# Autodesk Inventor assembly: metabotV2
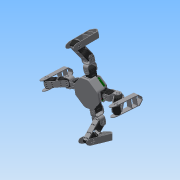
[picture p0: Inventor's stored thumbnail of the model, 180x180]
Saved by Autodesk Inventor 2015 (Build 190159000, 159)
## iProperties
Created: 2014-03-07
Part Number: metabotV2
Document SubType Name: Assembly
Designer: Grégoire
Author: Grégoire
## Documents named in this file (14)
- C:\Users\Gregwar\Desktop\Metabot\3d\autodesk\metabotV2.iam
- C:\Users\Gregwar\Desktop\Metabot\3d\autodesk\models\motor.ipt
- C:\Users\Gregwar\Desktop\Metabot\3d\autodesk\models\arm.ipt
- C:\Users\Gregwar\Desktop\Metabot\3d\autodesk\models\counter_arm.ipt
- C:\Users\Gregwar\Desktop\Metabot\3d\autodesk\parts\u.ipt
- C:\Users\Gregwar\Desktop\Metabot\3d\autodesk\parts\side.ipt
- C:\Users\Gregwar\Desktop\Metabot\3d\autodesk\parts\leg.ipt
- C:\Users\Gregwar\Desktop\Metabot\3d\autodesk\parts\bottom.ipt
- C:\Users\Gregwar\Desktop\Metabot\3d\autodesk\renfort.ipt
- C:\Users\Gregwar\Desktop\Metabot\3d\autodesk\models\x_board.ipt
- C:\Users\Gregwar\Desktop\Metabot\3d\autodesk\fix_top.ipt
- C:\Users\Gregwar\Desktop\Metabot\3d\autodesk\parts\magnet.ipt
- C:\Users\Gregwar\Desktop\Metabot\3d\autodesk\parts\head.ipt
- C:\Users\Gregwar\Desktop\Metabot\3d\autodesk\parts\top.ipt
## Components (66 placed, 13 different names)
1. motor:4 — Affleurement:2, Affleurement:4, Affleurement:5, Placage:211, Placage:217, Placage:218
2. arm:4 — Placage:167
3. counter_arm:4
4. u:3
5. u:4 — Placage:167
6. motor:5
7. arm:5
8. counter_arm:5
9. side:3
10. side:4
11. motor:6
12. arm:6
13. counter_arm:6
14. leg:2
15. motor:7 — Affleurement:3, Affleurement:4, Placage:215, Placage:216, Placage:223, Placage:224, Placage:225, Placage:241, Placage:242, Placage:243
16. arm:7
17. counter_arm:7 — Placage:168
18. u:5
19. u:6 — Placage:168
20. motor:8
21. arm:8
22. counter_arm:8
23. side:5
24. side:6
25. motor:9
26. arm:9
27. counter_arm:9
28. leg:3
29. motor:10 — Affleurement:1, Affleurement:2, Affleurement:5, Placage:197, Placage:212, Placage:219
30. arm:10
31. counter_arm:10 — Placage:169
32. u:7
33. u:8 — Placage:169
34. motor:11
35. arm:11
36. counter_arm:11
37. side:7
38. side:8
39. motor:12
40. arm:12
41. counter_arm:12
42. leg:4
43. renfort:1 — Placage:197
44. x_board:1 — Placage:221, Placage:222, Placage:226
45. bottom:1 — Placage:211, Placage:212, Placage:213, Placage:214, Placage:215, Placage:216, Placage:217, Placage:218, Placage:219, Placage:221, Placage:222, Placage:226
46. fix_top:1 — Placage:223, Placage:224, Placage:225, Placage:227, Placage:228, Placage:229, Placage:230, Placage:231, Placage:232, Placage:233, Placage:234, Placage:235, Placage:236, Placage:237, Placage:238, Placage:240
47. magnet:1 — Placage:227, Placage:228, Placage:229, Affleurement:6, Placage:244, Placage:245
48. magnet:2 — Placage:230, Placage:231, Placage:232, Affleurement:8, Placage:248, Placage:249, Placage:253
49. magnet:3 — Placage:233, Placage:234, Placage:235, Affleurement:7, Placage:246, Placage:247
50. magnet:4 — Placage:236, Placage:237, Placage:238, Placage:239, Affleurement:6, Affleurement:7, Affleurement:8, Placage:250, Placage:251
51. head:2 — Placage:239, Placage:240, Placage:252, Placage:254
52. top:1 — Placage:241, Placage:242, Placage:243, Placage:244, Placage:245, Placage:246, Placage:247, Placage:248, Placage:249, Placage:250, Placage:251, Placage:252, Placage:253, Placage:254
53. u:1 — Placage:7, Placage:8, Placage:9, Placage:14, Placage:15
54. u:2 — Placage:6, Placage:7, Placage:8, Placage:9, Placage:164, Placage:166
55. side:1 — Placage:19, Placage:20, Placage:21, Placage:26, Placage:27, Placage:28
56. side:2 — Placage:16, Placage:17, Placage:18
57. leg:1 — Placage:29, Placage:30
58. motor:1 — Placage:1, Placage:2, Placage:3, Placage:4, Affleurement:1, Affleurement:3, Placage:213, Placage:214
59. arm:1 — Placage:3, Placage:4, Placage:6, Placage:166
60. counter_arm:1 — Placage:1, Placage:2, Placage:164
61. motor:2 — Placage:16, Placage:17, Placage:18, Placage:19, Placage:20, Placage:21
62. arm:2 — Placage:15
63. counter_arm:2 — Placage:14
64. motor:3 — Placage:26, Placage:27, Placage:28
65. arm:3 — Placage:29, Placage:30
66. counter_arm:3
## Relationships (173: Mate 165, Flush 8)
- Placage:1 [Mate]: motor:1 ↔ counter_arm:1
- Placage:2 [Mate]: motor:1 ↔ counter_arm:1
- Placage:3 [Mate]: motor:1 ↔ arm:1
- Placage:4 [Mate]: motor:1 ↔ arm:1
- Placage:6 [Mate]: u:2 ↔ arm:1
- Placage:7 [Mate]: u:1 ↔ u:2
- Placage:8 [Mate]: u:1 ↔ u:2
- Placage:9 [Mate]: u:1 ↔ u:2
- [Mate]: motor:2 ↔ counter_arm:2
- [Mate]: motor:2 ↔ counter_arm:2
- [Mate]: motor:2 ↔ arm:2
- [Mate]: motor:2 ↔ arm:2
- Placage:14 [Mate]: u:1 ↔ counter_arm:2
- Placage:15 [Mate]: u:1 ↔ arm:2
- Placage:16 [Mate]: side:2 ↔ motor:2
- Placage:17 [Mate]: side:2 ↔ motor:2
- Placage:18 [Mate]: side:2 ↔ motor:2
- Placage:19 [Mate]: side:1 ↔ motor:2
- Placage:20 [Mate]: side:1 ↔ motor:2
- Placage:21 [Mate]: side:1 ↔ motor:2
- [Mate]: motor:3 ↔ counter_arm:3
- [Mate]: motor:3 ↔ counter_arm:3
- [Mate]: motor:3 ↔ arm:3
- [Mate]: motor:3 ↔ arm:3
- Placage:26 [Mate]: side:1 ↔ motor:3
- Placage:27 [Mate]: side:1 ↔ motor:3
- Placage:28 [Mate]: side:1 ↔ motor:3
- Placage:29 [Mate]: leg:1 ↔ arm:3
- Placage:30 [Mate]: leg:1 ↔ arm:3
- [Mate]: motor:4 ↔ counter_arm:4
- [Mate]: motor:4 ↔ counter_arm:4
- [Mate]: motor:4 ↔ arm:4
- [Mate]: motor:4 ↔ arm:4
- [Mate]: arm:4 ↔ u:4
- [Mate]: u:3 ↔ u:4
- [Mate]: u:3 ↔ u:4
- [Mate]: u:3 ↔ u:4
- [Mate]: motor:5 ↔ counter_arm:5
- [Mate]: motor:5 ↔ counter_arm:5
- [Mate]: motor:5 ↔ arm:5
- [Mate]: motor:5 ↔ arm:5
- [Mate]: u:3 ↔ counter_arm:5
- [Mate]: u:3 ↔ arm:5
- [Mate]: motor:5 ↔ side:4
- [Mate]: motor:5 ↔ side:4
- [Mate]: motor:5 ↔ side:4
- [Mate]: motor:5 ↔ side:3
- [Mate]: motor:5 ↔ side:3
- [Mate]: motor:5 ↔ side:3
- [Mate]: motor:6 ↔ counter_arm:6
- [Mate]: motor:6 ↔ counter_arm:6
- [Mate]: motor:6 ↔ arm:6
- [Mate]: motor:6 ↔ arm:6
- [Mate]: side:3 ↔ motor:6
- [Mate]: side:3 ↔ motor:6
- [Mate]: side:3 ↔ motor:6
- [Mate]: arm:6 ↔ leg:2
- [Mate]: arm:6 ↔ leg:2
- [Mate]: motor:7 ↔ counter_arm:7
- [Mate]: motor:7 ↔ counter_arm:7
- [Mate]: motor:7 ↔ arm:7
- [Mate]: motor:7 ↔ arm:7
- [Mate]: arm:7 ↔ u:6
- [Mate]: u:5 ↔ u:6
- [Mate]: u:5 ↔ u:6
- [Mate]: u:5 ↔ u:6
- [Mate]: motor:8 ↔ counter_arm:8
- [Mate]: motor:8 ↔ counter_arm:8
- [Mate]: motor:8 ↔ arm:8
- [Mate]: motor:8 ↔ arm:8
- [Mate]: u:5 ↔ counter_arm:8
- [Mate]: u:5 ↔ arm:8
- [Mate]: motor:8 ↔ side:6
- [Mate]: motor:8 ↔ side:6
- [Mate]: motor:8 ↔ side:6
- [Mate]: motor:8 ↔ side:5
- [Mate]: motor:8 ↔ side:5
- [Mate]: motor:8 ↔ side:5
- [Mate]: motor:9 ↔ counter_arm:9
- [Mate]: motor:9 ↔ counter_arm:9
- [Mate]: motor:9 ↔ arm:9
- [Mate]: motor:9 ↔ arm:9
- [Mate]: side:5 ↔ motor:9
- [Mate]: side:5 ↔ motor:9
- [Mate]: side:5 ↔ motor:9
- [Mate]: arm:9 ↔ leg:3
- [Mate]: arm:9 ↔ leg:3
- [Mate]: motor:10 ↔ counter_arm:10
- [Mate]: motor:10 ↔ counter_arm:10
- [Mate]: motor:10 ↔ arm:10
- [Mate]: motor:10 ↔ arm:10
- [Mate]: arm:10 ↔ u:8
- [Mate]: u:7 ↔ u:8
- [Mate]: u:7 ↔ u:8
- [Mate]: u:7 ↔ u:8
- [Mate]: motor:11 ↔ counter_arm:11
- [Mate]: motor:11 ↔ counter_arm:11
- [Mate]: motor:11 ↔ arm:11
- [Mate]: motor:11 ↔ arm:11
- [Mate]: u:7 ↔ counter_arm:11
- [Mate]: u:7 ↔ arm:11
- [Mate]: motor:11 ↔ side:8
- [Mate]: motor:11 ↔ side:8
- [Mate]: motor:11 ↔ side:8
- [Mate]: motor:11 ↔ side:7
- [Mate]: motor:11 ↔ side:7
- [Mate]: motor:11 ↔ side:7
- [Mate]: motor:12 ↔ counter_arm:12
- [Mate]: motor:12 ↔ counter_arm:12
- [Mate]: motor:12 ↔ arm:12
- [Mate]: motor:12 ↔ arm:12
- [Mate]: side:7 ↔ motor:12
- [Mate]: side:7 ↔ motor:12
- [Mate]: side:7 ↔ motor:12
- [Mate]: arm:12 ↔ leg:4
- [Mate]: arm:12 ↔ leg:4
- Placage:164 [Mate]: u:2 ↔ counter_arm:1
- Placage:166 [Mate]: u:2 ↔ arm:1
- Placage:167 [Mate]: arm:4 ↔ u:4
- Placage:168 [Mate]: counter_arm:7 ↔ u:6
- Placage:169 [Mate]: counter_arm:10 ↔ u:8
- Affleurement:1 [Flush]: motor:10 ↔ motor:1
- Affleurement:2 [Flush]: motor:4 ↔ motor:10
- Affleurement:3 [Flush]: motor:7 ↔ motor:1
- Affleurement:4 [Flush]: motor:4 ↔ motor:7
- Affleurement:5 [Flush]: motor:4 ↔ motor:10
- Placage:197 [Mate]: motor:10 ↔ renfort:1
- Placage:211 [Mate]: motor:4 ↔ bottom:1
- Placage:212 [Mate]: motor:10 ↔ bottom:1
- Placage:213 [Mate]: bottom:1 ↔ motor:1
- Placage:214 [Mate]: bottom:1 ↔ motor:1
- Placage:215 [Mate]: motor:7 ↔ bottom:1
- Placage:216 [Mate]: motor:7 ↔ bottom:1
- Placage:217 [Mate]: motor:4 ↔ bottom:1
- Placage:218 [Mate]: motor:4 ↔ bottom:1
- Placage:219 [Mate]: motor:10 ↔ bottom:1
- Placage:221 [Mate]: x_board:1 ↔ bottom:1
- Placage:222 [Mate]: x_board:1 ↔ bottom:1
- Placage:223 [Mate]: motor:7 ↔ fix_top:1
- Placage:224 [Mate]: motor:7 ↔ fix_top:1
- Placage:225 [Mate]: motor:7 ↔ fix_top:1
- Placage:226 [Mate]: x_board:1 ↔ bottom:1
- Placage:227 [Mate]: fix_top:1 ↔ magnet:1
- Placage:228 [Mate]: fix_top:1 ↔ magnet:1
- Placage:229 [Mate]: fix_top:1 ↔ magnet:1
- Placage:230 [Mate]: fix_top:1 ↔ magnet:2
- Placage:231 [Mate]: fix_top:1 ↔ magnet:2
- Placage:232 [Mate]: fix_top:1 ↔ magnet:2
- Placage:233 [Mate]: fix_top:1 ↔ magnet:3
- Placage:234 [Mate]: fix_top:1 ↔ magnet:3
- Placage:235 [Mate]: fix_top:1 ↔ magnet:3
- Placage:236 [Mate]: fix_top:1 ↔ magnet:4
- Placage:237 [Mate]: fix_top:1 ↔ magnet:4
- Placage:238 [Mate]: fix_top:1 ↔ magnet:4
- Placage:239 [Mate]: magnet:4 ↔ head:2
- Placage:240 [Mate]: fix_top:1 ↔ head:2
- Placage:241 [Mate]: motor:7 ↔ top:1
- Placage:242 [Mate]: motor:7 ↔ top:1
- Placage:243 [Mate]: motor:7 ↔ top:1
- Affleurement:6 [Flush]: magnet:1 ↔ magnet:4
- Affleurement:7 [Flush]: magnet:3 ↔ magnet:4
- Affleurement:8 [Flush]: magnet:2 ↔ magnet:4
- Placage:244 [Mate]: magnet:1 ↔ top:1
- Placage:245 [Mate]: magnet:1 ↔ top:1
- Placage:246 [Mate]: magnet:3 ↔ top:1
- Placage:247 [Mate]: magnet:3 ↔ top:1
- Placage:248 [Mate]: magnet:2 ↔ top:1
- Placage:249 [Mate]: magnet:2 ↔ top:1
- Placage:250 [Mate]: magnet:4 ↔ top:1
- Placage:251 [Mate]: magnet:4 ↔ top:1
- Placage:252 [Mate]: head:2 ↔ top:1
- Placage:253 [Mate]: magnet:2 ↔ top:1
- Placage:254 [Mate]: head:2 ↔ top:1
## Named parameters: d25_d0 = 0 mm, d26_d1 = 0 mm, d27_d2 = 0 mm, d28_d3 = 0 mm, d37_d0 = 0 mm, d38_d1 = 0 mm, d39_d2 = 0 mm, d40_d3 = 0 mm, d52_d0 = 0 mm, d53_d1 = 0 mm, d54_d2 = 0 mm, d55_d3 = 0 mm, d57_d21 = 0 mm, d58_d22 = 0 mm, d59_d23 = 0 mm, d60_d24 = 0 mm, d61_d25_d0 = 0 mm, d62_d26_d1 = 0 mm, d63_d27_d2 = 0 mm, d64_d28_d3 = 0 mm, d65_d29 = 0 mm, d66_d30 = 0 mm, d67_d31 = 0 mm, d68_d32 = 0 mm, d69_d33 = 0 mm, d70_d34 = 0 mm, d71_d35 = 0 mm, d72_d36 = 0 mm, d73_d37_d0 = 0 mm, d74_d38_d1 = 0 mm, d75_d39_d2 = 0 mm, d76_d40_d3 = 0 mm, d77_d41 = 0 mm, d78_d42 = 0 mm, d79_d43 = 0 mm, d80_d44 = 0 mm, d81_d45 = 0 mm, d82_d0 = 0 mm, d83_d1 = 0 mm, d84_d2 = 0 mm, d85_d3 = 0 mm, d87_d21 = 0 mm, d88_d22 = 0 mm, d89_d23 = 0 mm, d90_d24 = 0 mm, d91_d25_d0 = 0 mm, d92_d26_d1 = 0 mm, d93_d27_d2 = 0 mm, d94_d28_d3 = 0 mm, d95_d29 = 0 mm, d96_d30 = 0 mm, d97_d31 = 0 mm, d98_d32 = 0 mm, d99_d33 = 0 mm, d100_d34 = 0 mm, d101_d35 = 0 mm, d102_d36 = 0 mm, d103_d37_d0 = 0 mm, d104_d38_d1 = 0 mm, d105_d39_d2 = 0 mm, d106_d40_d3 = 0 mm, d107_d41 = 0 mm, d108_d42 = 0 mm, d109_d43 = 0 mm, d110_d44 = 0 mm, d111_d45 = 0 mm, d112_d0 = 0 mm, d113_d1 = 0 mm, d114_d2 = 0 mm, d115_d3 = 0 mm, d117_d21 = 0 mm, d118_d22 = 0 mm, d119_d23 = 0 mm, d120_d24 = 0 mm, d121_d25_d0 = 0 mm, d122_d26_d1 = 0 mm, d123_d27_d2 = 0 mm, d124_d28_d3 = 0 mm, d125_d29 = 0 mm, d126_d30 = 0 mm, d127_d31 = 0 mm, d128_d32 = 0 mm, d129_d33 = 0 mm, d130_d34 = 0 mm, d131_d35 = 0 mm, d132_d36 = 0 mm, d133_d37_d0 = 0 mm, d134_d38_d1 = 0 mm, d135_d39_d2 = 0 mm, d136_d40_d3 = 0 mm, d137_d41 = 0 mm, d138_d42 = 0 mm, d139_d43 = 0 mm, d140_d44 = 0 mm, d141_d45 = 0 mm
